# Autodesk Inventor assembly: Schweiss Baugruppe
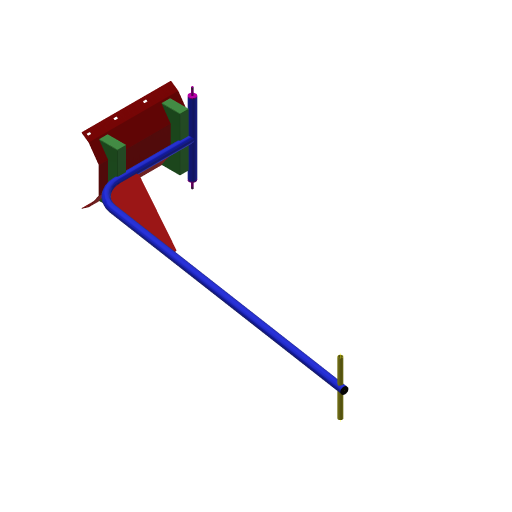
[picture p0: Inventor's stored thumbnail of the model, 512x512]
Saved by Autodesk Inventor 2023.2 (Build 272271000, 271)
## iProperties
Created: 2023-02-05
Part Number: Schweiss Baugruppe
Material: Generisch
Document SubType Name: Weldment
Designer: Raoul Messerli
Weld Material: Welded Aluminum-6061
Author: Raoul Messerli
## Documents named in this file (9)
- E:\GitHub\Pflanzenwagen\40_Realisieren\20_Inventor\40_Baugruppen\Schweiss Baugruppe.iam
- E:\GitHub\Pflanzenwagen\40_Realisieren\20_Inventor\30_Fertigungsteile\Blech1.ipt
- E:\GitHub\Pflanzenwagen\40_Realisieren\20_Inventor\30_Fertigungsteile\Halteblech.ipt
- E:\GitHub\Pflanzenwagen\40_Realisieren\20_Inventor\30_Fertigungsteile\Hebel.ipt
- E:\GitHub\Pflanzenwagen\40_Realisieren\20_Inventor\30_Fertigungsteile\Achse.ipt
- E:\GitHub\Pflanzenwagen\40_Realisieren\20_Inventor\30_Fertigungsteile\Rad Aufnahme.ipt
- E:\GitHub\Pflanzenwagen\40_Realisieren\20_Inventor\30_Fertigungsteile\Deckel.ipt
- E:\GitHub\Pflanzenwagen\40_Realisieren\20_Inventor\30_Fertigungsteile\Griff.ipt
- E:\GitHub\Pflanzenwagen\40_Realisieren\20_Inventor\30_Fertigungsteile\Keil.ipt
## Components (10 placed, 8 different names)
1. Blech1:1 — Fluchtend:1, Passend:1, Passend:2, Passend:3, Passend:4, Fluchtend:2, Fluchtend:3
2. Halteblech:1 — Passend:4, Passend:5, Fluchtend:3, Tangential:1
3. Halteblech:2 — Passend:3, Passend:6, Fluchtend:2, Passend:7
4. Hebel:1 — Passend:7, Fluchtend:4, Passend:8, Passend:13, Passend:14, Passend:15, Tangential:2, Tangential:3
5. Achse:2 — Passend:8, Fluchtend:5, Tangential:1, Passend:9, Passend:10, Passend:11, Passend:12
6. Rad Aufnahme:1 — Passend:9, Passend:10
7. Rad Aufnahme:2 — Passend:11, Passend:12
8. Deckel:1 — Passend:13, Passend:14
9. Griff:1 — Passend:15, Fluchtend:6
10. Keil:1 — Passend:16, Tangential:2, Tangential:3
## Relationships (25: Mate 16, Flush 6, Tangent 3)
- Fluchtend:1 [Flush]: Blech1:1
- Passend:1 [Mate]: Blech1:1
- Passend:2 [Mate]: Blech1:1
- Passend:3 [Mate]: Blech1:1 ↔ Halteblech:2
- Passend:4 [Mate]: Blech1:1 ↔ Halteblech:1
- Passend:5 [Mate]: Halteblech:1
- Passend:6 [Mate]: Halteblech:2
- Fluchtend:2 [Flush] (100 mm): Blech1:1 ↔ Halteblech:2
- Fluchtend:3 [Flush] (800 mm): Blech1:1 ↔ Halteblech:1
- Passend:7 [Mate]: Halteblech:2 ↔ Hebel:1
- Fluchtend:4 [Flush]: Hebel:1
- Passend:8 [Mate]: Hebel:1 ↔ Achse:2
- Fluchtend:5 [Flush] (400 mm): Achse:2
- Tangential:1: Halteblech:1 ↔ Achse:2
- Passend:9 [Mate]: Achse:2 ↔ Rad Aufnahme:1
- Passend:10 [Mate]: Achse:2 ↔ Rad Aufnahme:1
- Passend:11 [Mate]: Achse:2 ↔ Rad Aufnahme:2
- Passend:12 [Mate]: Achse:2 ↔ Rad Aufnahme:2
- Passend:13 [Mate]: Hebel:1 ↔ Deckel:1
- Passend:14 [Mate]: Hebel:1 ↔ Deckel:1
- Passend:15 [Mate]: Hebel:1 ↔ Griff:1
- Fluchtend:6 [Flush]: Griff:1
- Passend:16 [Mate]: Keil:1
- Tangential:2: Hebel:1 ↔ Keil:1
- Tangential:3: Hebel:1 ↔ Keil:1
## Named parameters: sa_0 = 250000
note: some values were not read from the file. Shown as the stored number, unit unknown: "sa_0".
